# Autodesk Inventor assembly: side c
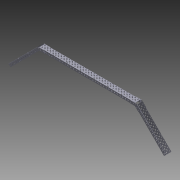
[picture p0: Inventor's stored thumbnail of the model, 180x180]
Saved by Autodesk Inventor 2015 (Build 190159000, 159)
## iProperties
Created: 2015-09-05
Part Number: side c
Document SubType Name: Assembly
Designer: myps3_000
Author: myps3_000
## Documents named in this file (4)
- C:\Users\myps3_000\Desktop\dev\vex\custome\side c.iam
- C:\Users\myps3_000\Desktop\dev\vex\Metal\C-Channels\C-Channel 1x2x1x35.ipt
- C:\Users\myps3_000\Desktop\dev\vex\Metal\Gussets\45 Degree Gusset.ipt
- C:\Users\myps3_000\Desktop\dev\vex\Metal\C-Channels\C-Channel 1x2x1x15.ipt
## Components (7 placed, 3 different names)
1. C-Channel 1x2x1x35:2 — Insert:1, Insert:2, Insert:5, Insert:6, Insert:7, Insert:8, Insert:11
2. 45 Degree Gusset:2 — Insert:1, Insert:2, Insert:3, Insert:4
3. 45 Degree Gusset:8 — Insert:5, Insert:6
4. 45 Degree Gusset:9 — Insert:7, Insert:8, Insert:9, Insert:10
5. 45 Degree Gusset:10 — Insert:11, Insert:12
6. C-Channel 1x2x1x15:1 — Insert:9, Insert:10, Insert:12
7. C-Channel 1x2x1x15:4 — Insert:3, Insert:4
## Relationships (12: Insert 12)
- Insert:1: C-Channel 1x2x1x35:2 ↔ 45 Degree Gusset:2
- Insert:2: C-Channel 1x2x1x35:2 ↔ 45 Degree Gusset:2
- Insert:3: 45 Degree Gusset:2 ↔ C-Channel 1x2x1x15:4
- Insert:4: 45 Degree Gusset:2 ↔ C-Channel 1x2x1x15:4
- Insert:5: C-Channel 1x2x1x35:2 ↔ 45 Degree Gusset:8
- Insert:6: C-Channel 1x2x1x35:2 ↔ 45 Degree Gusset:8
- Insert:7: C-Channel 1x2x1x35:2 ↔ 45 Degree Gusset:9
- Insert:8: C-Channel 1x2x1x35:2 ↔ 45 Degree Gusset:9
- Insert:9: 45 Degree Gusset:9 ↔ C-Channel 1x2x1x15:1
- Insert:10: 45 Degree Gusset:9 ↔ C-Channel 1x2x1x15:1
- Insert:11: C-Channel 1x2x1x35:2 ↔ 45 Degree Gusset:10
- Insert:12: 45 Degree Gusset:10 ↔ C-Channel 1x2x1x15:1
